# Autodesk Inventor assembly: FullAssem
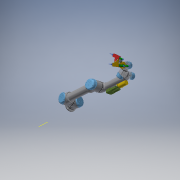
[picture p0: Inventor's stored thumbnail of the model, 180x180]
Saved by Autodesk Inventor 2018 (Build 220112000, 112)
## iProperties
Created: 2020-04-08
Part Number: FullAssem
Document SubType Name: Assembly
Designer: Jesse R-B
Author: Jesse R-B
## Documents named in this file (6)
- C:\Users\Jesse R-B\Documents\Inventor\400\V2\V3\FullAssem.iam
- C:\Users\Jesse R-B\Documents\Inventor\400\ur5-5.snapshot.3\UR5Assem.iam
- C:\Users\Jesse R-B\Documents\Inventor\400\V2\V3\Assembly2.iam
- C:\Users\Jesse R-B\Documents\Inventor\400\V2\V3\ReducedLargeSyrgine.ipt
- C:\Users\Jesse R-B\Documents\Inventor\400\V2\V3\reducedLargeSyrginePlunger.ipt
- C:\Users\Jesse R-B\Documents\Inventor\400\V2\V3\actuator assem.iam
## Components (5 placed, 5 different names)
1. UR5Assem:1 [sub-assembly] — Mate:1, Mate:2, Mate:3, Mate:4, Mate:5, Flush:1, Mate:7, Mate:9
2. Assembly2:1 [sub-assembly] — Mate:1, Mate:2, Mate:3
3. ReducedLargeSyrgine:1 — Mate:4, Mate:5, Flush:1, Mate:6, Flush:2
4. reducedLargeSyrginePlunger:1 — Mate:6, Flush:2, Mate:8, Mate:10
5. actuator assem:1 [sub-assembly] — Mate:7, Mate:8, Mate:9, Mate:10
## Relationships (12: Mate 10, Flush 2)
- Mate:1: UR5Assem:1 ↔ Assembly2:1
- Mate:2: UR5Assem:1 ↔ Assembly2:1
- Mate:3: UR5Assem:1 ↔ Assembly2:1
- Mate:4: UR5Assem:1 ↔ ReducedLargeSyrgine:1
- Mate:5 (63.5 mm): UR5Assem:1 ↔ ReducedLargeSyrgine:1
- Flush:1: UR5Assem:1 ↔ ReducedLargeSyrgine:1
- Mate:6: ReducedLargeSyrgine:1 ↔ reducedLargeSyrginePlunger:1
- Flush:2: ReducedLargeSyrgine:1 ↔ reducedLargeSyrginePlunger:1
- Mate:7: UR5Assem:1 ↔ actuator assem:1
- Mate:8: reducedLargeSyrginePlunger:1 ↔ actuator assem:1
- Mate:9 (63.5 mm): UR5Assem:1 ↔ actuator assem:1
- Mate:10: reducedLargeSyrginePlunger:1 ↔ actuator assem:1
